# Autodesk Inventor assembly: Inner
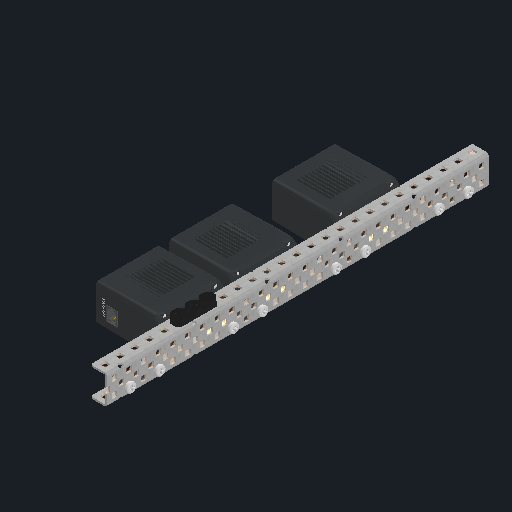
[picture p0: Inventor's stored thumbnail of the model, 512x512]
Saved by Autodesk Inventor 2025 (Build 290162000, 162)
## iProperties
Created: 2024-12-17
Part Number: Inner
Document SubType Name: Assembly
Designer: avere
Author: Averey Ku
## Documents named in this file (9)
- D:\VEX\High Stakes\CAD\V4\Chassis\Drivebay Right\Inner.iam
- D:\VEX\High Stakes\CAD\V4\Chassis\Drivebay Right\Alu C 1x2x1x26.ipt
- D:\VEX\High Stakes\CAD\V4\Chassis\Drivebay Right\Nylon Standoff .875.ipt
- D:\VEX\High Stakes\CAD\V4\Chassis\Drivebay Right\V5 Motor.ipt
- D:\VEX\High Stakes\CAD\V4\Chassis\Drivebay Right\NScrew Pan Head Threaded .500.ipt
- D:\VEX\High Stakes\CAD\V4\Chassis\Drivebay Right\Nut Nylon Thread-Forming.ipt
- D:\VEX\High Stakes\CAD\V4\Chassis\Drivebay Right\Bearing Flat Low Profile.ipt
- D:\VEX\High Stakes\CAD\ROBOPROS-CAD-Inventor\Structure\Hardware\Screw Nylon - Pan Head\NScrew Pan Head Threaded .250.ipt
- D:\VEX\High Stakes\CAD\ROBOPROS-CAD-Inventor\Motion\Shaft LS\Bearing Flat.ipt
## Components (29 placed, 8 different names)
1. Alu C 1x2x1x26:1 — Flush:3, Flush:2, Flush:1, Insert:1, Insert:10, Mate:3, Mate:2, Insert:7, Insert:9, Insert:10, Mate:4, Insert:12, Insert:13, Mate:5
2. Nylon Standoff .875:1 — Insert:1
3. Nylon Standoff .875:2
4. NScrew Pan Head Threaded .250:1 — Insert:9
5. Bearing Flat:1 — Insert:10, Mate:4
6. Nut Nylon Thread-Forming:9 — Insert:13
7. V5 Motor:3 — Insert:12, Mate:5
8. V5 Motor:1 — Mate:2, Insert:7
9. V5 Motor:2
10. NScrew Pan Head Threaded .500:1 — Mate:3, Insert:9
11. NScrew Pan Head Threaded .500:2 — Insert:10, Insert:8
12. Nut Nylon Thread-Forming:1 — Insert:3
13. Nut Nylon Thread-Forming:2 — Insert:2
14. Bearing Flat Low Profile:1 — Insert:2, Insert:3, Insert:8, Insert:9
15. NScrew Pan Head Threaded .500:3
16. NScrew Pan Head Threaded .500:4
17. Nut Nylon Thread-Forming:3
18. Nut Nylon Thread-Forming:4
19. Bearing Flat Low Profile:2
20. NScrew Pan Head Threaded .500:5
21. NScrew Pan Head Threaded .500:6
22. Nut Nylon Thread-Forming:5
23. Nut Nylon Thread-Forming:6
24. Bearing Flat Low Profile:3
25. NScrew Pan Head Threaded .500:7
26. NScrew Pan Head Threaded .500:8
27. Nut Nylon Thread-Forming:7
28. Nut Nylon Thread-Forming:8
29. Bearing Flat Low Profile:4
## Component patterns: (2 elements, first: V5 Motor:1), (4 elements, first: NScrew Pan Head Threaded .500:1 + NScrew Pan Head Threaded .500:2 + Nut Nylon Thread-Forming:1 + Nut Nylon Thread-Forming:2 + Bearing Flat Low Profile:1)
## Relationships (18: Insert 11, Mate 5, Flush 2)
- Flush:3 (-12.7 mm): Alu C 1x2x1x26:1
- Flush:2 (-7.9375 mm): Alu C 1x2x1x26:1
- Flush:1 [Mate] (-165.1 mm): Alu C 1x2x1x26:1
- Insert:1: Alu C 1x2x1x26:1 ↔ Nylon Standoff .875:1
- Insert:2 (1.27 mm): Nut Nylon Thread-Forming:2 ↔ Bearing Flat Low Profile:1
- Insert:3 (1.27 mm): Nut Nylon Thread-Forming:1 ↔ Bearing Flat Low Profile:1
- Insert:10: Alu C 1x2x1x26:1 ↔ NScrew Pan Head Threaded .500:2
- Insert:8 (1.5875 mm): NScrew Pan Head Threaded .500:2 ↔ Bearing Flat Low Profile:1
- Mate:3: Alu C 1x2x1x26:1 ↔ NScrew Pan Head Threaded .500:1
- Insert:9 (1.5875 mm): NScrew Pan Head Threaded .500:1 ↔ Bearing Flat Low Profile:1
- Mate:2: Alu C 1x2x1x26:1 ↔ V5 Motor:1
- Insert:7: Alu C 1x2x1x26:1 ↔ V5 Motor:1
- Insert:9: Alu C 1x2x1x26:1 ↔ NScrew Pan Head Threaded .250:1
- Insert:10: Alu C 1x2x1x26:1 ↔ Bearing Flat:1
- Mate:4: Alu C 1x2x1x26:1 ↔ Bearing Flat:1
- Insert:12: Alu C 1x2x1x26:1 ↔ V5 Motor:3
- Insert:13: Alu C 1x2x1x26:1 ↔ Nut Nylon Thread-Forming:9
- Mate:5: Alu C 1x2x1x26:1 ↔ V5 Motor:3
